# Autodesk Inventor assembly: Owen Cabinet
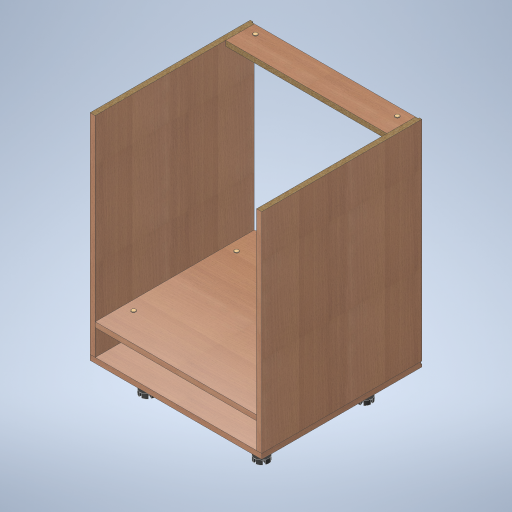
[picture p0: Inventor's stored thumbnail of the model, 512x512]
Saved by Autodesk Inventor 2024 (Build 280153000, 153)
## iProperties
RuleStatus: InUse
Created: 2017-01-19
Part Number: Owen Cabinet
Document SubType Name: Assembly
Designer: SvetlanaB
Author: SvetlanaB
## Documents named in this file (17)
- C:\W4INV 2024 Design\iBOX LIBRARY\Kitchen\Standing Cabinets\Owen Cabinet\Owen Cabinet.iam
- C:\W4INV 2024 Design\iBOX LIBRARY\Kitchen\Standing Cabinets\Owen Cabinet\Top panel.ipt
- C:\W4INV 2024 Design\iBOX LIBRARY\Kitchen\Standing Cabinets\Owen Cabinet\Right panel.ipt
- C:\W4INV 2024 Design\iBOX LIBRARY\Kitchen\Standing Cabinets\Owen Cabinet\Bottom panel.ipt
- C:\W4INV 2024 Design\iBOX LIBRARY\Kitchen\Standing Cabinets\Owen Cabinet\Left panel.ipt
- C:\W4INV 2024 Design\iBOX LIBRARY\Kitchen\Standing Cabinets\Owen Cabinet\Bottom panel copy.ipt
- C:\W4INV 2024 Design\iBOX LIBRARY\Kitchen\Standing Cabinets\Owen Cabinet\Back panel.ipt
- C:\W4INV 2024 Design\_LIBRARY\Supports and legs\Legs\ADJUSTABLE LEG\Adjustable leg  BT18 clip included.ipt
- C:\W4INV 2024 Design\_LIBRARY\Supports and legs\Legs\ADJUSTABLE LEG\Adjustable leg  BT18.ipt
- C:\W4INV 2024 Design\_LIBRARY\Fixed joints\Confirmat\CONFIRMAT\Confirmat L50 NB T18 PB T 18.ipt
- C:\W4INV 2024 Design\iBOX LIBRARY\Kitchen\Standing Cabinets\Owen Cabinet\Owen Cabinet.ipt
- C:\W4INV 2024 Design\_LIBRARY\Fixed joints\Confirmat\CONFIRMAT\Confirmat L50 & Cap D10 NB T18 PB T 18.ipt
- C:\W4INV 2024 Design\_LIBRARY\Fixed joints\Minifix joint\MINIFIX D15 v2\Minifix D15 & Dowel L34 & Cap D15 PB T18 RH.ipt
- C:\W4INV 2024 Design\_LIBRARY\Fixed joints\Minifix joint\MINIFIX D15 v2\Minifix D15 & Dowel L34 & Cap D15 PB T18 LH.ipt
- C:\W4INV 2023 Design\LIBRARY\Fixed joints\Confirmat\CONFIRMAT.ipt
- C:\W4INV 2023 Design\LIBRARY\Fixed joints\Minifix joint\MINIFIX D15 v2.ipt
- C:\W4INV 2023 Design\LIBRARY\Supports and legs\Legs\ADJUSTABLE LEG.ipt
## Components (21 placed, 13 different names)
1. @Skeleton
2. Top panel:1 — Flush:22, Pillar Board Side Plane :1, Pillar Board Side Plane :2
3. Right panel:1 — Flush:2, Pillar Board Side Plane:5, Pillar Board Side Plane:7, Nestled Board Plane:2, Nestled Board Plane:4, Nestled Board Plane:10
4. Bottom panel:1 — Flush:1, Bottom board Plane:1, Bottom board Plane:4, Bottom board Plane:2, Front (Angle) Plane:1, Bottom board Plane:3, Front (Angle) Plane:2, Nestled Board Plane:5, Nestled Board Plane:6, Nestled Board Plane:7, Nestled Board Plane:8
5. Left panel:1 — Flush:3, Flush:5, Flush:6, Pillar Board Side Plane:6, Pillar Board Side Plane:8, Nestled Board Plane:1, Nestled Board Plane:3, Nestled Board Plane:9
6. Bottom panel copy:1 — Pillar Board Side Plane :3, Pillar Board Side Plane :4, Pillar Board Side Plane :5, Pillar Board Side Plane :6
7. Back panel:1 — Flush:4
8. Adjustable leg  BT18:1 — Bottom board Plane:1, Axis Plane:1, Axis2 Plane:1
9. Adjustable leg  BT18:4 — Bottom board Plane:4, Axis Plane:4, Axis2 Plane:4
10. Adjustable leg  BT18 clip included:5 — Axis2 Plane:2, Bottom board Plane:2, Axis Plane:2, Front (Angle) Plane:1
11. Adjustable leg  BT18 clip included:6 — Axis2 Plane:3, Bottom board Plane:3, Axis Plane:3, Front (Angle) Plane:2
12. Confirmat L50 & Cap D10 NB T18 PB T 18:11 — Axis Plane:9, Pillar Board Side Plane:5, Nestled Board Plane:5
13. Confirmat L50 NB T18 PB T 18:12 — Axis Plane:10, Pillar Board Side Plane:6, Nestled Board Plane:6
14. Confirmat L50 NB T18 PB T 18:13 — Axis Plane:11, Pillar Board Side Plane:7, Nestled Board Plane:7
15. Confirmat L50 NB T18 PB T 18:14 — Axis Plane:12, Pillar Board Side Plane:8, Nestled Board Plane:8
16. Minifix D15 & Dowel L34 & Cap D15 PB T18 RH:1 — Nestled Board Plane:1, Axis Plane:5, Pillar Board Side Plane :1
17. Minifix D15 & Dowel L34 & Cap D15 PB T18 LH:2 — Nestled Board Plane:2, Axis Plane:6, Pillar Board Side Plane :2
18. Minifix D15 & Dowel L34 & Cap D15 PB T18 RH:3 — Axis Plane:7, Nestled Board Plane:3, Pillar Board Side Plane :3
19. Minifix D15 & Dowel L34 & Cap D15 PB T18 LH:4 — Axis Plane:8, Nestled Board Plane:4, Pillar Board Side Plane :4
20. Minifix D15 & Dowel L34 & Cap D15 PB T18 LH:5 — Axis Plane:13, Nestled Board Plane:9, Pillar Board Side Plane :5
21. Minifix D15 & Dowel L34 & Cap D15 PB T18 RH:6 — Axis Plane:14, Nestled Board Plane:10, Pillar Board Side Plane :6
## Relationships (51: Mate 32, Flush 17, Angle 2)
- Flush:1 (-100 mm): Bottom panel:1
- Flush:2 (-100 mm): Right panel:1
- Flush:3 (-100 mm): Left panel:1
- Flush:4 (-100 mm): Back panel:1
- Bottom board Plane:1 [Mate]: Bottom panel:1 ↔ Adjustable leg  BT18:1
- Axis Plane:1 [Mate]: Adjustable leg  BT18:1
- Axis2 Plane:1 [Mate]: Adjustable leg  BT18:1
- Bottom board Plane:4 [Mate]: Bottom panel:1 ↔ Adjustable leg  BT18:4
- Axis Plane:4 [Mate]: Adjustable leg  BT18:4
- Axis2 Plane:4 [Mate]: Adjustable leg  BT18:4
- Flush:5 (-64 mm): Left panel:1
- Flush:6 (-64 mm): Left panel:1
- Axis2 Plane:2 [Mate]: Adjustable leg  BT18 clip included:5
- Bottom board Plane:2 [Mate]: Bottom panel:1 ↔ Adjustable leg  BT18 clip included:5
- Axis Plane:2 [Mate]: Adjustable leg  BT18 clip included:5
- Front (Angle) Plane:1 [Angle] (0 deg): Bottom panel:1 ↔ Adjustable leg  BT18 clip included:5
- Axis2 Plane:3 [Mate]: Adjustable leg  BT18 clip included:6
- Bottom board Plane:3 [Mate]: Bottom panel:1 ↔ Adjustable leg  BT18 clip included:6
- Axis Plane:3 [Mate]: Adjustable leg  BT18 clip included:6
- Front (Angle) Plane:2 [Angle] (0 deg): Bottom panel:1 ↔ Adjustable leg  BT18 clip included:6
- Axis Plane:9 [Mate]: Confirmat L50 & Cap D10 NB T18 PB T 18:11
- Pillar Board Side Plane:5 [Mate] (-9 mm): Right panel:1 ↔ Confirmat L50 & Cap D10 NB T18 PB T 18:11
- Nestled Board Plane:5 [Flush]: Bottom panel:1 ↔ Confirmat L50 & Cap D10 NB T18 PB T 18:11
- Axis Plane:10 [Mate]: Confirmat L50 NB T18 PB T 18:12
- Pillar Board Side Plane:6 [Mate] (-9 mm): Left panel:1 ↔ Confirmat L50 NB T18 PB T 18:12
- Nestled Board Plane:6 [Flush]: Bottom panel:1 ↔ Confirmat L50 NB T18 PB T 18:12
- Axis Plane:11 [Mate]: Confirmat L50 NB T18 PB T 18:13
- Pillar Board Side Plane:7 [Mate] (-9 mm): Right panel:1 ↔ Confirmat L50 NB T18 PB T 18:13
- Nestled Board Plane:7 [Flush]: Bottom panel:1 ↔ Confirmat L50 NB T18 PB T 18:13
- Axis Plane:12 [Mate]: Confirmat L50 NB T18 PB T 18:14
- Pillar Board Side Plane:8 [Mate] (-9 mm): Left panel:1 ↔ Confirmat L50 NB T18 PB T 18:14
- Nestled Board Plane:8 [Flush]: Bottom panel:1 ↔ Confirmat L50 NB T18 PB T 18:14
- Flush:22 (-30 mm): Top panel:1
- Nestled Board Plane:1 [Mate]: Left panel:1 ↔ Minifix D15 & Dowel L34 & Cap D15 PB T18 RH:1
- Axis Plane:5 [Mate]: Minifix D15 & Dowel L34 & Cap D15 PB T18 RH:1
- Nestled Board Plane:2 [Mate]: Right panel:1 ↔ Minifix D15 & Dowel L34 & Cap D15 PB T18 LH:2
- Axis Plane:6 [Mate]: Minifix D15 & Dowel L34 & Cap D15 PB T18 LH:2
- Pillar Board Side Plane :1 [Flush] (18 mm): Top panel:1 ↔ Minifix D15 & Dowel L34 & Cap D15 PB T18 RH:1
- Pillar Board Side Plane :2 [Flush] (18 mm): Top panel:1 ↔ Minifix D15 & Dowel L34 & Cap D15 PB T18 LH:2
- Axis Plane:7 [Mate]: Minifix D15 & Dowel L34 & Cap D15 PB T18 RH:3
- Nestled Board Plane:3 [Mate]: Left panel:1 ↔ Minifix D15 & Dowel L34 & Cap D15 PB T18 RH:3
- Pillar Board Side Plane :3 [Flush] (18 mm): Bottom panel copy:1 ↔ Minifix D15 & Dowel L34 & Cap D15 PB T18 RH:3
- Axis Plane:8 [Mate]: Minifix D15 & Dowel L34 & Cap D15 PB T18 LH:4
- Nestled Board Plane:4 [Mate]: Right panel:1 ↔ Minifix D15 & Dowel L34 & Cap D15 PB T18 LH:4
- Pillar Board Side Plane :4 [Flush] (18 mm): Bottom panel copy:1 ↔ Minifix D15 & Dowel L34 & Cap D15 PB T18 LH:4
- Axis Plane:13 [Mate]: Minifix D15 & Dowel L34 & Cap D15 PB T18 LH:5
- Nestled Board Plane:9 [Mate]: Left panel:1 ↔ Minifix D15 & Dowel L34 & Cap D15 PB T18 LH:5
- Pillar Board Side Plane :5 [Flush] (18 mm): Bottom panel copy:1 ↔ Minifix D15 & Dowel L34 & Cap D15 PB T18 LH:5
- Axis Plane:14 [Mate]: Minifix D15 & Dowel L34 & Cap D15 PB T18 RH:6
- Nestled Board Plane:10 [Mate]: Right panel:1 ↔ Minifix D15 & Dowel L34 & Cap D15 PB T18 RH:6
- Pillar Board Side Plane :6 [Flush] (18 mm): Bottom panel copy:1 ↔ Minifix D15 & Dowel L34 & Cap D15 PB T18 RH:6
## Named parameters: Panel_thickness = 18 mm, Space_for_drawer = 90 mm, Space_For_Owen_Facade = 632.999 mm, Space_For_Owen_Body = 605.999 mm
